# Autodesk Inventor assembly: VidPad PCB (2)
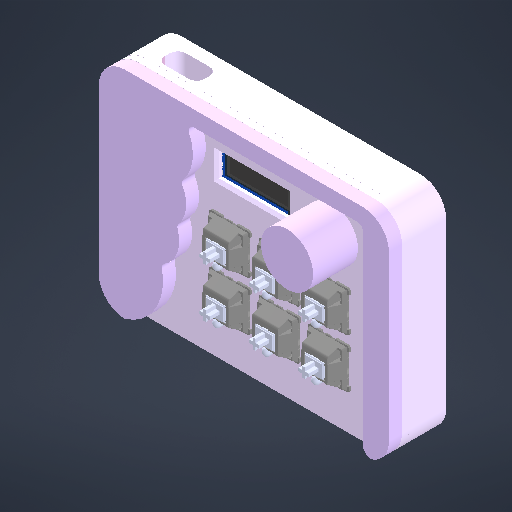
[picture p0: Inventor's stored thumbnail of the model, 512x512]
Saved by Autodesk Inventor 2026.2 (Build 302298000, 298)
## iProperties
Company: Kicad
Created: 2026-02-15
Part Number: VidPad PCB (2)
Description: KiCad electronic assembly
Document SubType Name: Assembly
Designer: bh
Authority: Unknown
Sending System: KiCad to STEP converter
Preprocessor: Open CASCADE STEP processor 7.8
Title: VidPad PCB.step
Author: Pcbnew
## Documents named in this file (15)
- C:\Users\bh\Downloads\VidPad-with-PCB.iam
- C:\Users\bh\Downloads\VidPad PCB (2)\VidPad PCB (2)\MX.iam
- C:\Users\bh\Downloads\VidPad PCB (2)\VidPad PCB (2)\æè½¬ç¼ç å¨.ipt
- C:\Users\bh\Downloads\VidPad PCB (2)\VidPad PCB (2)\0.91in OLED Module - Without Glass v1.iam
- C:\Users\bh\Downloads\VidPad PCB (2)\VidPad PCB (2)\D_DO-35_SOD27_P7.62mm_Horizontal.ipt
- C:\Users\bh\Downloads\VidPad PCB (2)\VidPad PCB (2)\VidPad PCB_copper.ipt
- C:\Users\bh\Downloads\VidPad PCB (2)\VidPad PCB (2)\VidPad PCB_silkscreen.ipt
- C:\Users\bh\Downloads\VidPad PCB (2)\VidPad PCB (2)\VidPad PCB_silkscreen_1.ipt
- C:\Users\bh\Downloads\VidPad PCB (2)\VidPad PCB (2)\VidPad PCB_soldermask.ipt
- C:\Users\bh\Downloads\VidPad PCB (2)\VidPad PCB (2)\VidPad PCB_soldermask_1.ipt
- C:\Users\bh\Downloads\VidPad PCB (2)\VidPad PCB (2)\VidPad PCB_PCB.ipt
- C:\Users\bh\Downloads\Top.ipt
- C:\Users\bh\Downloads\RotaryEncoderKnob.ipt
- C:\Users\bh\Downloads\Middle.ipt
- C:\Users\bh\Downloads\Bottom.ipt
## Components (24 placed, 24 different names)
1. 6 [sub-assembly]
2. 7 [sub-assembly]
3. 8 [sub-assembly] — Mate:1, Mate:2
4. 9 — Rotational:3
5. 10 [sub-assembly]
6. 11 [sub-assembly]
7. 31 [sub-assembly]
8. 32 [sub-assembly]
9. 33
10. 34
11. 35
12. 36
13. 37
14. 38
15. 39
16. 40
17. 41
18. 42
19. 43
20. 44
21. Top:1 — Rotational:5
22. RotaryEncoderKnob:1 — Rotational:3
23. Middle:1 — Mate:1, Mate:2, Rotational:4, Rotational:5
24. Bottom:1 — Rotational:4
## Relationships (5: RevoluteJoint 3, Mate 2)
- Rotational:3 [RevoluteJoint]: 9 ↔ RotaryEncoderKnob:1
- Mate:1 (0.2 mm): 8 ↔ Middle:1
- Mate:2 (0.2 mm): 8 ↔ Middle:1
- Rotational:4 [RevoluteJoint]: Middle:1 ↔ Bottom:1
- Rotational:5 [RevoluteJoint]: Top:1 ↔ Middle:1
